# Autodesk Inventor assembly: 35 напр
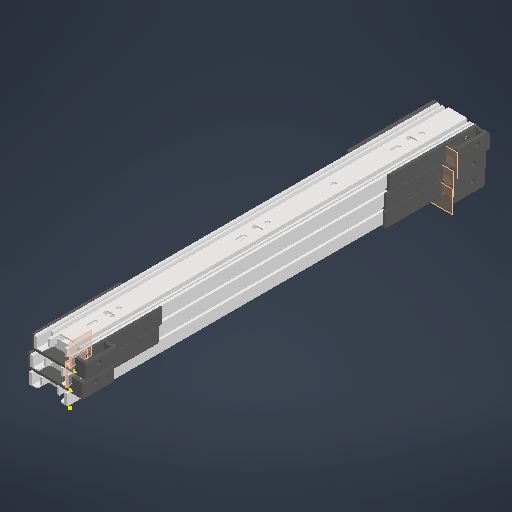
[picture p0: Inventor's stored thumbnail of the model, 512x512]
Saved by Autodesk Inventor 2025 (Build 290162000, 162)
## iProperties
Created: 2025-01-08
Part Number: 35 напр
Document SubType Name: Assembly
Designer: GameHD
Author: GameHD
## Documents named in this file (6)
- C:\Users\GameHD\Desktop\phantom 16950\35 напр.iam
- C:\Users\GameHD\Desktop\phantom 16950\3 часть направляшки 35.ipt
- C:\Users\GameHD\Desktop\phantom 16950\1 часть направляшки 35.ipt
- C:\Users\GameHD\Desktop\phantom 16950\2 часть направляшки 35.ipt
- C:\Users\GameHD\Desktop\phantom 16950\блоки\блоки.ipt
- C:\Users\GameHD\Desktop\phantom 16950\БЛОКИ С 3 ДЫРКАМИ\БЛОКИ С 3 ДЫРКАМИ копия.ipt
## Components (14 placed, 5 different names)
1. 3 часть направляшки 35:1 — Совмещение:2, Совмещение:3, Заподлицо:7, Совмещение:15
2. 2 часть направляшки 35:1 — Совмещение:1, Совмещение:2, Совмещение:3, Совмещение:4
3. 1 часть направляшки 35:1 — Совмещение:1, Совмещение:4, Совмещение:5, Совмещение:6, Заподлицо:3, Заподлицо:8
4. блоки:1 — Совмещение:11, Совмещение:12, Заподлицо:6, Заподлицо:7, Совмещение:15, Заподлицо:12
5. БЛОКИ С 3 ДЫРКАМИ копия:1 — Совмещение:5, Совмещение:6, Заподлицо:3
6. 3 часть направляшки 35:2 — Совмещение:24, Заподлицо:13
7. 2 часть направляшки 35:2
8. 1 часть направляшки 35:2 — Совмещение:11, Совмещение:12, Заподлицо:6, Совмещение:13, Совмещение:14, Заподлицо:8, Заподлицо:9
9. БЛОКИ С 3 ДЫРКАМИ копия:2 — Совмещение:13, Совмещение:14, Заподлицо:9
10. блоки:2 — Совмещение:24, Заподлицо:12, Заподлицо:13
11. 3 часть направляшки 35:3
12. 2 часть направляшки 35:3
13. 1 часть направляшки 35:3
14. БЛОКИ С 3 ДЫРКАМИ копия:3
## Relationships (33: Mate 24, Flush 9)
- Совмещение:1 [Mate]: 2 часть направляшки 35:1 ↔ 1 часть направляшки 35:1
- Совмещение:2 [Mate]: 3 часть направляшки 35:1 ↔ 2 часть направляшки 35:1
- Совмещение:3 [Mate] (2.5 mm): 3 часть направляшки 35:1 ↔ 2 часть направляшки 35:1
- Совмещение:4 [Mate] (1.25 mm): 2 часть направляшки 35:1 ↔ 1 часть направляшки 35:1
- Совмещение:5 [Mate]: 1 часть направляшки 35:1 ↔ БЛОКИ С 3 ДЫРКАМИ копия:1
- Совмещение:6 [Mate]: 1 часть направляшки 35:1 ↔ БЛОКИ С 3 ДЫРКАМИ копия:1
- Заподлицо:3 [Flush]: 1 часть направляшки 35:1 ↔ БЛОКИ С 3 ДЫРКАМИ копия:1
- [Mate]: 2 часть направляшки 35:2 ↔ 1 часть направляшки 35:2
- [Mate]: 3 часть направляшки 35:2 ↔ 2 часть направляшки 35:2
- [Mate] (2.5 mm): 3 часть направляшки 35:2 ↔ 2 часть направляшки 35:2
- [Mate] (1.25 mm): 2 часть направляшки 35:2 ↔ 1 часть направляшки 35:2
- Совмещение:11 [Mate]: блоки:1 ↔ 1 часть направляшки 35:2
- Совмещение:12 [Mate]: блоки:1 ↔ 1 часть направляшки 35:2
- Заподлицо:6 [Flush]: блоки:1 ↔ 1 часть направляшки 35:2
- Совмещение:13 [Mate]: 1 часть направляшки 35:2 ↔ БЛОКИ С 3 ДЫРКАМИ копия:2
- Совмещение:14 [Mate]: 1 часть направляшки 35:2 ↔ БЛОКИ С 3 ДЫРКАМИ копия:2
- Заподлицо:7 [Flush]: 3 часть направляшки 35:1 ↔ блоки:1
- Заподлицо:8 [Flush]: 1 часть направляшки 35:1 ↔ 1 часть направляшки 35:2
- Совмещение:15 [Mate]: 3 часть направляшки 35:1 ↔ блоки:1
- Заподлицо:9 [Flush]: 1 часть направляшки 35:2 ↔ БЛОКИ С 3 ДЫРКАМИ копия:2
- [Mate]: 2 часть направляшки 35:3 ↔ 1 часть направляшки 35:3
- [Mate]: 3 часть направляшки 35:3 ↔ 2 часть направляшки 35:3
- [Mate] (2.5 mm): 3 часть направляшки 35:3 ↔ 2 часть направляшки 35:3
- [Mate] (1.25 mm): 2 часть направляшки 35:3 ↔ 1 часть направляшки 35:3
- [Mate]: блоки:2 ↔ 1 часть направляшки 35:3
- [Mate]: блоки:2 ↔ 1 часть направляшки 35:3
- [Flush]: блоки:2 ↔ 1 часть направляшки 35:3
- [Mate]: 1 часть направляшки 35:3 ↔ БЛОКИ С 3 ДЫРКАМИ копия:3
- [Mate]: 1 часть направляшки 35:3 ↔ БЛОКИ С 3 ДЫРКАМИ копия:3
- [Flush]: 1 часть направляшки 35:3 ↔ БЛОКИ С 3 ДЫРКАМИ копия:3
- Совмещение:24 [Mate]: 3 часть направляшки 35:2 ↔ блоки:2
- Заподлицо:12 [Flush]: блоки:1 ↔ блоки:2
- Заподлицо:13 [Flush]: 3 часть направляшки 35:2 ↔ блоки:2
## Named parameters: d19_d8 = 0 mm, d20_d9 = 0 mm, d21_d10 = 2.5 mm, d22_d11 = 1.25 mm, d36_d19_d8 = 0 mm, d37_d20_d9 = 0 mm, d38_d21_d10 = 2.5 mm, d39_d22_d11 = 1.25 mm, d40_d25 = 0 mm, d41_d27 = 0 mm, d42_d28 = 0 mm, d43_d29 = 0 mm, d44_d30 = 0 mm, d45_d35 = 0 mm
